# Autodesk Inventor assembly: mini Cryostat FOOT3
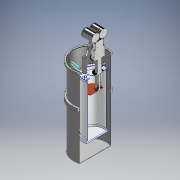
[picture p0: Inventor's stored thumbnail of the model, 180x180]
Saved by Autodesk Inventor 2018 (Build 220112000, 112)
## iProperties
Created: 2018-10-10
Part Number: mini Cryostat FOOT3
Document SubType Name: Assembly
Designer: Admin
Author: Admin
## Documents named in this file (11)
- C:\Users\freyja\Documents\Cryorefrigerator\CAD\mini Cryostat FOOT3.iam
- C:\Users\freyja\Documents\Cryorefrigerator\CAD\External Models\CH40415 24JUL14 C.ipt
- C:\Users\freyja\Documents\Cryorefrigerator\CAD\vacuum jacket long.ipt
- C:\Users\freyja\Documents\Cryorefrigerator\CAD\vacuum jacket.ipt
- C:\Users\freyja\Documents\Cryorefrigerator\CAD\Top Plate V2.2.ipt
- C:\Users\freyja\Documents\Cryorefrigerator\CAD\mini 55K stage.ipt
- C:\Users\freyja\Documents\Cryorefrigerator\CAD\still pipe standin.ipt
- C:\Users\freyja\Documents\Cryorefrigerator\CAD\foot type 3.iam
- C:\Users\freyja\Documents\Cryorefrigerator\CAD\2K8 stage mini.ipt
- C:\Users\freyja\Documents\Cryorefrigerator\CAD\foot type 2 length 2.iam
- C:\Users\freyja\Documents\Cryorefrigerator\CAD\Radiation Sheild 2K.ipt
## Components (20 placed, 10 different names)
1. Top Plate V2.2:1 — Mate:16, Mate:18, Mate:19, Mate:20, Mate:21, Mate:26, Mate:47, Mate:57, Mate:58, Mate:59, Mate:60, Mate:61, Mate:62, Mate:89, Mate:105, Mate:106
2. CH40415 24JUL14 C:1 — Mate:16, Mate:18, Mate:26, Mate:46, Flush:1
3. vacuum jacket long:1 — Mate:7, Mate:8, Mate:9
4. vacuum jacket:1 — Mate:7, Mate:8, Mate:9, Mate:19, Mate:20, Mate:21
5. mini 55K stage:1 — Mate:46, Mate:48, Flush:1, Mate:49, Mate:50, Mate:52, Mate:53, Mate:54, Mate:55, Mate:56, Mate:81, Mate:82, Mate:83, Mate:84, Mate:85, Mate:86, Mate:87, Mate:88, Mate:90, Mate:91, Mate:92, Mate:93, Mate:94, Mate:97, Mate:100, Mate:101, Mate:102, Mate:103, Mate:104
6. still pipe standin:1 — Mate:47, Mate:48, Mate:67
7. foot type 3:1 [sub-assembly] — Mate:58, Mate:89, Mate:97
8. foot type 3:2 [sub-assembly] — Mate:52, Mate:57, Mate:90
9. foot type 3:3 [sub-assembly] — Mate:53, Mate:60, Mate:92
10. foot type 3:4 [sub-assembly] — Mate:54, Mate:59, Mate:91
11. foot type 3:5 [sub-assembly] — Mate:50, Mate:62, Mate:94
12. foot type 3:6 [sub-assembly] — Mate:49, Mate:61, Mate:93
13. foot type 3:7 [sub-assembly] — Mate:55, Mate:103, Mate:105
14. foot type 3:8 [sub-assembly] — Mate:56, Mate:104, Mate:106
15. 2K8 stage mini:1 — Mate:67
16. foot type 2 length 2:1 [sub-assembly] — Mate:82, Mate:88
17. foot type 2 length 2:2 [sub-assembly] — Mate:81, Mate:85
18. foot type 2 length 2:3 [sub-assembly] — Mate:83, Mate:86
19. foot type 2 length 2:4 [sub-assembly] — Mate:84, Mate:87
20. Radiation Sheild 2K:1 — Mate:100, Mate:101, Mate:102
## Relationships (49: Mate 48, Flush 1)
- Mate:7: vacuum jacket long:1 ↔ vacuum jacket:1
- Mate:8: vacuum jacket long:1 ↔ vacuum jacket:1
- Mate:9: vacuum jacket long:1 ↔ vacuum jacket:1
- Mate:16: Top Plate V2.2:1 ↔ CH40415 24JUL14 C:1
- Mate:18: Top Plate V2.2:1 ↔ CH40415 24JUL14 C:1
- Mate:19: Top Plate V2.2:1 ↔ vacuum jacket:1
- Mate:20: Top Plate V2.2:1 ↔ vacuum jacket:1
- Mate:21: Top Plate V2.2:1 ↔ vacuum jacket:1
- Mate:26: Top Plate V2.2:1 ↔ CH40415 24JUL14 C:1
- Mate:46: CH40415 24JUL14 C:1 ↔ mini 55K stage:1
- Mate:47: Top Plate V2.2:1 ↔ still pipe standin:1
- Mate:48: mini 55K stage:1 ↔ still pipe standin:1
- Flush:1: CH40415 24JUL14 C:1 ↔ mini 55K stage:1
- Mate:49: mini 55K stage:1 ↔ foot type 3:6
- Mate:50: mini 55K stage:1 ↔ foot type 3:5
- Mate:52: mini 55K stage:1 ↔ foot type 3:2
- Mate:53: mini 55K stage:1 ↔ foot type 3:3
- Mate:54: mini 55K stage:1 ↔ foot type 3:4
- Mate:55: mini 55K stage:1 ↔ foot type 3:7
- Mate:56: mini 55K stage:1 ↔ foot type 3:8
- Mate:57: Top Plate V2.2:1 ↔ foot type 3:2
- Mate:58 (2.54 mm): Top Plate V2.2:1 ↔ foot type 3:1
- Mate:59: Top Plate V2.2:1 ↔ foot type 3:4
- Mate:60: Top Plate V2.2:1 ↔ foot type 3:3
- Mate:61: Top Plate V2.2:1 ↔ foot type 3:6
- Mate:62: Top Plate V2.2:1 ↔ foot type 3:5
- Mate:67: still pipe standin:1 ↔ 2K8 stage mini:1
- Mate:81: mini 55K stage:1 ↔ foot type 2 length 2:2
- Mate:82: mini 55K stage:1 ↔ foot type 2 length 2:1
- Mate:83: mini 55K stage:1 ↔ foot type 2 length 2:3
- Mate:84: mini 55K stage:1 ↔ foot type 2 length 2:4
- Mate:85: mini 55K stage:1 ↔ foot type 2 length 2:2
- Mate:86: mini 55K stage:1 ↔ foot type 2 length 2:3
- Mate:87: mini 55K stage:1 ↔ foot type 2 length 2:4
- Mate:88: mini 55K stage:1 ↔ foot type 2 length 2:1
- Mate:89: Top Plate V2.2:1 ↔ foot type 3:1
- Mate:90: mini 55K stage:1 ↔ foot type 3:2
- Mate:91: mini 55K stage:1 ↔ foot type 3:4
- Mate:92: mini 55K stage:1 ↔ foot type 3:3
- Mate:93: mini 55K stage:1 ↔ foot type 3:6
- Mate:94: mini 55K stage:1 ↔ foot type 3:5
- Mate:97: mini 55K stage:1 ↔ foot type 3:1
- Mate:100: mini 55K stage:1 ↔ Radiation Sheild 2K:1
- Mate:101: mini 55K stage:1 ↔ Radiation Sheild 2K:1
- Mate:102: mini 55K stage:1 ↔ Radiation Sheild 2K:1
- Mate:103: mini 55K stage:1 ↔ foot type 3:7
- Mate:104: mini 55K stage:1 ↔ foot type 3:8
- Mate:105: Top Plate V2.2:1 ↔ foot type 3:7
- Mate:106: Top Plate V2.2:1 ↔ foot type 3:8
